# Autodesk Inventor assembly: PCB Stack Concept V03 04
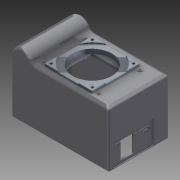
[picture p0: Inventor's stored thumbnail of the model, 180x180]
Saved by Autodesk Inventor 2015 (Build 190159000, 159)
## iProperties
Created: 2014-04-13
Part Number: PCB Stack Concept V03 04
Document SubType Name: Assembly
Designer: spichelh
Author: spichelh
## Documents named in this file (15)
- C:\Users\spichelh\Documents\GitHub\beta-hardware\Enclosure\Version 002\PCB Stack Concept V03 04.iam
- C:\Users\spichelh\Documents\GitHub\beta-hardware\Enclosure\Version 002\Cooler.ipt
- C:\Users\spichelh\Documents\GitHub\beta-hardware\Enclosure\Version 002\SFE-Host01.ipt
- C:\Users\spichelh\Documents\GitHub\beta-hardware\Enclosure\Version 002\SFE-ProcessingBoard01.ipt
- C:\Users\spichelh\Documents\GitHub\beta-hardware\Enclosure\Version 002\PCBModuleLeft02.ipt
- C:\Users\spichelh\Documents\GitHub\beta-hardware\Enclosure\Version 002\BetaBoard01.ipt
- C:\Users\spichelh\Documents\GitHub\beta-hardware\Enclosure\Version 002\Imported Components\Zynq_Z010_uZed_F_Prod\Zynq_Z010_uZed_F_Prod.ipt
- C:\Users\spichelh\Documents\GitHub\beta-hardware\Enclosure\Version 002\PowerPCB01.ipt
- C:\Users\spichelh\Documents\GitHub\beta-hardware\Enclosure\Version 002\Imported Components\Samtec-PCIE-036-02-D-F-TH\Samtec-PCIE-036-02-D-F-TH.ipt
- C:\Users\spichelh\Documents\GitHub\beta-hardware\Enclosure\Version 002\SensorCooler01.ipt
- C:\Users\spichelh\Documents\GitHub\beta-hardware\Enclosure\Skeleton_E-mount\Imported Components\CMV12000v1\CMV12000v1.ipt
- C:\Users\spichelh\Documents\GitHub\beta-hardware\Enclosure\Skeleton_E-mount\Imported Components\Sensormount_CMV12000-H\Sensormount_CMV12000-H.ipt
- C:\Users\spichelh\Documents\GitHub\beta-hardware\Enclosure\Version 002\threaded-rod01.ipt
- C:\Users\spichelh\Documents\GitHub\beta-hardware\Enclosure\Version 002\Simple3DPrintEnclosure01.ipt
- C:\Users\spichelh\Documents\Inventor\Content Center Files\R2015\en-US\ANSI B18.6.4(04)\ANSI B18.6.4 - 4-24 - 0,375(1) B IA.ipt
## Components (22 placed, 14 different names)
1. Cooler:1 — Flush:120, Flush:121, Mate:162
2. SFE-Host01:1 — Mate:73, Flush:48, Flush:49, Flush:121, Mate:162, Flush:125, Flush:126, Mate:163
3. SFE-ProcessingBoard01:1 — Mate:73, Flush:48, Flush:49, Flush:109, Mate:134, Flush:112, Mate:136, Flush:123, Flush:124, Mate:159
4. PCBModuleLeft02:1 — Flush:109, Mate:134, Flush:113, Flush:114
5. BetaBoard01:1 — Mate:135, Flush:110, Flush:111, Flush:112, Mate:136, Flush:113, Flush:114, Mate:137, Mate:138, Flush:115, Flush:116, Mate:142, Mate:143, Flush:117, Flush:120
6. Zynq_Z010_uZed_F_Prod:1 — Mate:131, Flush:107, Flush:108
7. PowerPCB01:1 — Mate:131, Flush:107, Flush:108, Mate:135, Flush:110, Flush:111
8. Samtec-PCIE-036-02-D-F-TH:1 — Mate:137, Mate:138, Flush:115, Flush:116
9. Samtec-PCIE-036-02-D-F-TH:2 — Mate:142, Mate:143, Flush:117
10. SensorCooler01:1
11. PCBModuleLeft02:2 — Flush:123, Flush:124, Mate:159
12. CMV12000v1:1 — Flush:125, Flush:126, Mate:163, Mate:164, Mate:165, Mate:166
13. Sensormount_CMV12000-H:1 — Mate:164, Mate:165, Mate:166, Mate:167, Flush:127, Mate:168, Mate:169, Mate:170, Mate:171, Flush:128, Flush:129, Mate:172, Flush:130, Flush:131
14. threaded-rod01:1 — Mate:168, Flush:128
15. threaded-rod01:2 — Mate:169, Flush:129
16. threaded-rod01:3 — Mate:170, Mate:171
17. threaded-rod01:4 — Mate:172, Flush:130
18. Simple3DPrintEnclosure01:1 — Flush:131, Mate:173, Mate:174, Mate:175, Mate:176
19. Cross Recessed 100° Flat Countersunk Head Tapping Screw - Type B - Type IA - Inch No. 4 - 24 -  3/8:1 — Mate:173
20. Cross Recessed 100° Flat Countersunk Head Tapping Screw - Type B - Type IA - Inch No. 4 - 24 -  3/8:2 — Mate:174
21. Cross Recessed 100° Flat Countersunk Head Tapping Screw - Type B - Type IA - Inch No. 4 - 24 -  3/8:3 — Mate:175
22. Cross Recessed 100° Flat Countersunk Head Tapping Screw - Type B - Type IA - Inch No. 4 - 24 -  3/8:4 — Mate:176
## Relationships (49: Mate 25, Flush 24)
- Mate:73: SFE-Host01:1 ↔ SFE-ProcessingBoard01:1
- Flush:48: SFE-Host01:1 ↔ SFE-ProcessingBoard01:1
- Flush:49: SFE-Host01:1 ↔ SFE-ProcessingBoard01:1
- Mate:131 (7 mm): Zynq_Z010_uZed_F_Prod:1 ↔ PowerPCB01:1
- Flush:107: Zynq_Z010_uZed_F_Prod:1 ↔ PowerPCB01:1
- Flush:108: Zynq_Z010_uZed_F_Prod:1 ↔ PowerPCB01:1
- Flush:109: SFE-ProcessingBoard01:1 ↔ PCBModuleLeft02:1
- Mate:134 (1 mm): SFE-ProcessingBoard01:1 ↔ PCBModuleLeft02:1
- Mate:135 (5 mm): BetaBoard01:1 ↔ PowerPCB01:1
- Flush:110: BetaBoard01:1 ↔ PowerPCB01:1
- Flush:111: BetaBoard01:1 ↔ PowerPCB01:1
- Flush:112: SFE-ProcessingBoard01:1 ↔ BetaBoard01:1
- Mate:136: SFE-ProcessingBoard01:1 ↔ BetaBoard01:1
- Flush:113: PCBModuleLeft02:1 ↔ BetaBoard01:1
- Flush:114: PCBModuleLeft02:1 ↔ BetaBoard01:1
- Mate:137: BetaBoard01:1 ↔ Samtec-PCIE-036-02-D-F-TH:1
- Mate:138: BetaBoard01:1 ↔ Samtec-PCIE-036-02-D-F-TH:1
- Flush:115: BetaBoard01:1 ↔ Samtec-PCIE-036-02-D-F-TH:1
- Flush:116 (1.4908 mm): BetaBoard01:1 ↔ Samtec-PCIE-036-02-D-F-TH:1
- Mate:142: BetaBoard01:1 ↔ Samtec-PCIE-036-02-D-F-TH:2
- Mate:143: BetaBoard01:1 ↔ Samtec-PCIE-036-02-D-F-TH:2
- Flush:117 (2.0906 mm): BetaBoard01:1 ↔ Samtec-PCIE-036-02-D-F-TH:2
- Flush:120 (30 mm): Cooler:1 ↔ BetaBoard01:1
- Flush:121 (2 mm): Cooler:1 ↔ SFE-Host01:1
- Flush:123: SFE-ProcessingBoard01:1 ↔ PCBModuleLeft02:2
- Flush:124: SFE-ProcessingBoard01:1 ↔ PCBModuleLeft02:2
- Mate:159 (2 mm): SFE-ProcessingBoard01:1 ↔ PCBModuleLeft02:2
- Mate:162 (1 mm): Cooler:1 ↔ SFE-Host01:1
- Flush:125 (11.875 mm): SFE-Host01:1 ↔ CMV12000v1:1
- Flush:126 (5.175 mm): SFE-Host01:1 ↔ CMV12000v1:1
- Mate:163 (3 mm): SFE-Host01:1 ↔ CMV12000v1:1
- Mate:164: CMV12000v1:1 ↔ Sensormount_CMV12000-H:1
- Mate:165 (0.05 mm): CMV12000v1:1 ↔ Sensormount_CMV12000-H:1
- Mate:166: CMV12000v1:1 ↔ Sensormount_CMV12000-H:1
- Mate:167: Sensormount_CMV12000-H:1
- Flush:127: Sensormount_CMV12000-H:1
- Mate:168: Sensormount_CMV12000-H:1 ↔ threaded-rod01:1
- Mate:169: Sensormount_CMV12000-H:1 ↔ threaded-rod01:2
- Mate:170: Sensormount_CMV12000-H:1 ↔ threaded-rod01:3
- Mate:171: Sensormount_CMV12000-H:1 ↔ threaded-rod01:3
- Flush:128: Sensormount_CMV12000-H:1 ↔ threaded-rod01:1
- Flush:129: Sensormount_CMV12000-H:1 ↔ threaded-rod01:2
- Mate:172: Sensormount_CMV12000-H:1 ↔ threaded-rod01:4
- Flush:130: Sensormount_CMV12000-H:1 ↔ threaded-rod01:4
- Flush:131: Sensormount_CMV12000-H:1 ↔ Simple3DPrintEnclosure01:1
- Mate:173: Simple3DPrintEnclosure01:1 ↔ Cross Recessed 100° Flat Countersunk Head Tapping Screw - Type B - Type IA - Inch No. 4 - 24 -  3/8:1
- Mate:174: Simple3DPrintEnclosure01:1 ↔ Cross Recessed 100° Flat Countersunk Head Tapping Screw - Type B - Type IA - Inch No. 4 - 24 -  3/8:2
- Mate:175: Simple3DPrintEnclosure01:1 ↔ Cross Recessed 100° Flat Countersunk Head Tapping Screw - Type B - Type IA - Inch No. 4 - 24 -  3/8:3
- Mate:176: Simple3DPrintEnclosure01:1 ↔ Cross Recessed 100° Flat Countersunk Head Tapping Screw - Type B - Type IA - Inch No. 4 - 24 -  3/8:4
